# Autodesk Inventor assembly: End_Effector_Calibration_tool
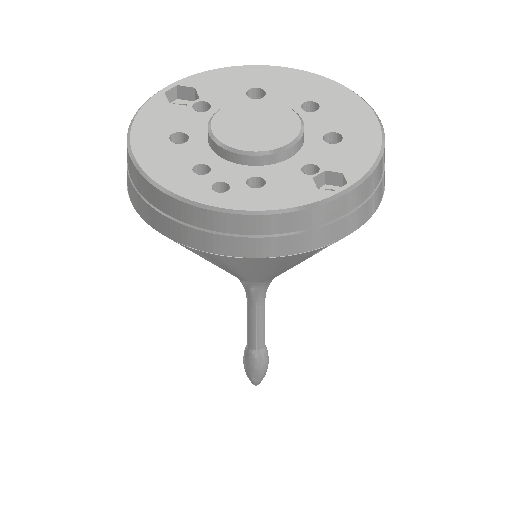
[picture p0: Inventor's stored thumbnail of the model, 512x512]
Saved by Autodesk Inventor 2025.2 (Build 292293000, 293)
## iProperties
Created: 2025-05-22
Part Number: End_Effector_Calibration_tool
Document SubType Name: Assembly
Designer: Marcu
Author: Marcu
## Documents named in this file (4)
- C:\Users\Marcu\Documents\GitHub\Semesterprojekt-2025\3D filer\End_Effector_Calibration_tool.iam
- C:\Users\Marcu\Downloads\End-effector calibration tool_End-effector calibration tool v9_Top Flange.ipt
- C:\Users\Marcu\Downloads\End-effector calibration tool_End-effector calibration tool v9_Pointer tool.ipt
- C:\Users\Marcu\Downloads\End-effector calibration tool_End-effector calibration tool v9_Bottom Flange.ipt
## Components (3 placed, 3 different names)
1. End-effector calibration tool_End-effector calibration tool v9_Top Flange:1 — Mate:1
2. End-effector calibration tool_End-effector calibration tool v9_Pointer tool:1 — Mate:2
3. End-effector calibration tool_End-effector calibration tool v9_Bottom Flange:1 — Mate:1, Mate:2
## Relationships (2: Mate 2)
- Mate:1: End-effector calibration tool_End-effector calibration tool v9_Top Flange:1 ↔ End-effector calibration tool_End-effector calibration tool v9_Bottom Flange:1
- Mate:2: End-effector calibration tool_End-effector calibration tool v9_Pointer tool:1 ↔ End-effector calibration tool_End-effector calibration tool v9_Bottom Flange:1
